# Autodesk Inventor assembly: BC-100002
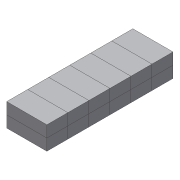
[picture p0: Inventor's stored thumbnail of the model, 180x180]
Saved by Autodesk Inventor 2016 (Build 200138000, 138)
## iProperties
Created: 2015-09-23
Part Number: BC-100002
Document SubType Name: Assembly
Designer: Reinaldo.Basílio
Author: Reinaldo.Basílio
## Documents named in this file (2)
- D:\ARQ\Basilio\LNLS-2\Anel\Dipolos\BC-3T\Dipolo 3T e 1T\Prototipo 1\Projeto Mecanico\BC-100002.iam
- D:\ARQ\Basilio\LNLS-2\Anel\Dipolos\BC-3T\Dipolo 3T e 1T\Prototipo 1\Projeto Mecanico\NdFeB.ipt
## Components (12 placed, 1 different names)
1. NdFeB:1
2. NdFeB:2
3. NdFeB:3
4. NdFeB:4
5. NdFeB:5
6. NdFeB:6
7. NdFeB:7
8. NdFeB:8
9. NdFeB:9
10. NdFeB:10
11. NdFeB:11
12. NdFeB:12
## Component patterns: (12 elements, first: NdFeB:1)
